# Autodesk Inventor assembly: Assembly1
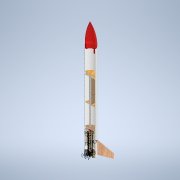
[picture p0: Inventor's stored thumbnail of the model, 180x180]
Saved by Autodesk Inventor 2020 (Build 240168000, 168)
## iProperties
Created: 2021-10-16
Part Number: Assembly1
Document SubType Name: Assembly
Designer: Carlos
Mass: 1446.2 g
Surface Area: 5943.29 cm^2
Volume: 695.431 cm^3
Density: 2.07957 g/cm^3
Author: Carlos
## Documents named in this file (7)
- \\CARLOS-PC\Shared\UdeA\Diseño Conceptual\CAD Cohete\CAD 2 - copia\Cohete\Ensamble Cohete.iam
- \\CARLOS-PC\Shared\UdeA\Diseño Conceptual\CAD Cohete\CAD 2 - copia\Cohete\Tubo Central.ipt
- \\CARLOS-PC\Shared\UdeA\Diseño Conceptual\CAD Cohete\CAD 2 - copia\Cohete\Aletas.ipt
- \\CARLOS-PC\Shared\UdeA\Diseño Conceptual\CAD Cohete\CAD 2 - copia\Anillos\CAD\Ensamble MDF.iam
- \\CARLOS-PC\Shared\UdeA\Diseño Conceptual\CAD Cohete\CAD 2 - copia\Sistema de Eyección\CAD\Sistema de Eyección 1.iam
- \\CARLOS-PC\Shared\UdeA\Diseño Conceptual\CAD Cohete\CAD 2 - copia\Ojiva\Ojiva Tangente.ipt
- \\CARLOS-PC\Shared\UdeA\Diseño Conceptual\CAD Cohete\CAD 2 - copia\Sistema de Eyección\CAD\Soporte Eyección.ipt
## Components (9 placed, 6 different names)
1. Tubo Central:1 — Mate:1, Mate:6, Mate:7, Mate:8, Mate:11, Mate:12, Mate:13
2. Ensamble MDF:1 [sub-assembly] — Mate:6, Mate:7
3. Sistema de Eyección 1:1 [sub-assembly] — Mate:8
4. Ojiva Tangente:1 — Mate:12, Mate:13
5. Soporte Eyección:1 — Mate:11
6. Aletas:1 — Mate:1
7. Aletas:2
8. Aletas:3
9. Aletas:4
## Component patterns: (4 elements, first: Aletas:1)
## Relationships (7: Mate 7)
- Mate:1: Tubo Central:1 ↔ Aletas:1
- Mate:6: Tubo Central:1 ↔ Ensamble MDF:1
- Mate:7: Tubo Central:1 ↔ Ensamble MDF:1
- Mate:8: Tubo Central:1 ↔ Sistema de Eyección 1:1
- Mate:11: Tubo Central:1 ↔ Soporte Eyección:1
- Mate:12: Tubo Central:1 ↔ Ojiva Tangente:1
- Mate:13: Tubo Central:1 ↔ Ojiva Tangente:1
